# Autodesk Inventor assembly: DriveTrainSide
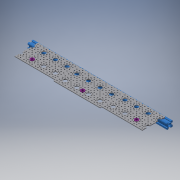
[picture p0: Inventor's stored thumbnail of the model, 180x180]
Saved by Autodesk Inventor 2018 (Build 220112000, 112)
## iProperties
Created: 2017-10-27
Part Number: DriveTrainSide
Document SubType Name: Assembly
Designer: ball
Author: ball
## Documents named in this file (6)
- C:\FTC\2017Robot\DriveTrainSide.iam
- C:\FTC\Actobotics\585 parts\585002_5_25x3_0.ipt
- C:\FTC\Actobotics\585 parts\585002_6_0x3_22.ipt
- C:\FTC\Actobotics\535 parts\535198.ipt
- C:\FTC\Actobotics\565 parts\565062.ipt
- C:\FTC\Actobotics\585 parts\585718.ipt
## Components (11 placed, 5 different names)
1. 585002_5_25x3_0:1 — Flush:2, Mate:10, Mate:14, Mate:15, Flush:6, Mate:18, Mate:21, Mate:22, Mate:25
2. 585002_5_25x3_0:2 — Mate:11, Flush:4, Flush:5, Mate:12, Mate:17, Flush:7, Mate:28, Mate:29, Mate:32
3. 585002_6_0x3_22:1 — Flush:2, Mate:10, Mate:11, Flush:4, Flush:5, Mate:13, Flush:6, Mate:16
4. 535198:2 — Mate:14, Mate:15
5. 535198:3 — Mate:13, Mate:16
6. 535198:4 — Mate:12, Mate:17
7. 565062:1 — Mate:18, Flush:7, Mate:19, Mate:20, Mate:23, Mate:24, Mate:26, Mate:27, Mate:30, Mate:31
8. 585718:1 — Mate:19, Mate:20, Mate:21, Mate:22
9. 585718:2 — Mate:26, Mate:27, Mate:28, Mate:29
10. 585718:3 — Mate:23, Mate:24, Mate:25
11. 585718:4 — Mate:30, Mate:31, Mate:32
## Relationships (28: Mate 23, Flush 5)
- Flush:2: 585002_5_25x3_0:1 ↔ 585002_6_0x3_22:1
- Mate:10: 585002_5_25x3_0:1 ↔ 585002_6_0x3_22:1
- Mate:11: 585002_5_25x3_0:2 ↔ 585002_6_0x3_22:1
- Flush:4: 585002_5_25x3_0:2 ↔ 585002_6_0x3_22:1
- Flush:5: 585002_5_25x3_0:2 ↔ 585002_6_0x3_22:1
- Mate:12: 585002_5_25x3_0:2 ↔ 535198:4
- Mate:13: 585002_6_0x3_22:1 ↔ 535198:3
- Mate:14: 585002_5_25x3_0:1 ↔ 535198:2
- Mate:15: 585002_5_25x3_0:1 ↔ 535198:2
- Flush:6: 585002_5_25x3_0:1 ↔ 585002_6_0x3_22:1
- Mate:16: 585002_6_0x3_22:1 ↔ 535198:3
- Mate:17: 585002_5_25x3_0:2 ↔ 535198:4
- Mate:18: 585002_5_25x3_0:1 ↔ 565062:1
- Flush:7 (-19.05 mm): 585002_5_25x3_0:2 ↔ 565062:1
- Mate:19: 565062:1 ↔ 585718:1
- Mate:20 (0.0635 mm): 565062:1 ↔ 585718:1
- Mate:21: 585002_5_25x3_0:1 ↔ 585718:1
- Mate:22: 585002_5_25x3_0:1 ↔ 585718:1
- Mate:23: 565062:1 ↔ 585718:3
- Mate:24 (0.0635 mm): 565062:1 ↔ 585718:3
- Mate:25: 585002_5_25x3_0:1 ↔ 585718:3
- Mate:26: 565062:1 ↔ 585718:2
- Mate:27 (0.0635 mm): 565062:1 ↔ 585718:2
- Mate:28: 585002_5_25x3_0:2 ↔ 585718:2
- Mate:29: 585002_5_25x3_0:2 ↔ 585718:2
- Mate:30: 565062:1 ↔ 585718:4
- Mate:31 (0.0635 mm): 565062:1 ↔ 585718:4
- Mate:32: 585002_5_25x3_0:2 ↔ 585718:4
